# Autodesk Inventor assembly: Battery Rack Assembly
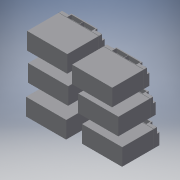
[picture p0: Inventor's stored thumbnail of the model, 180x180]
Saved by Autodesk Inventor 2019.4 (Build 234330000, 330)
## iProperties
Created: 2020-02-27
Part Number: Battery Rack Assembly
Document SubType Name: Assembly
Designer: admin
Author: admin
## Documents named in this file (2)
- C:\Users\admin\Desktop\FRC 2020 Engineering\GitHub\7738-2020\Pit Station Designs\battery rack\Battery Rack Assembly.iam
- C:\Users\admin\Desktop\FRC 2020 Engineering\GitHub\7738-2020\CAD\Battery.ipt
## Components (6 placed, 1 different names)
1. Battery:1 — Flush:1, Mate:1, Flush:5
2. Battery:2 — Flush:3, Mate:4, Flush:5
3. Battery:3 — Flush:3, Flush:4, Mate:3, Mate:4
4. Battery:4 — Flush:1, Flush:2, Mate:1, Mate:2
5. Battery:5 — Flush:4, Mate:3, Mate:5
6. Battery:6 — Flush:2, Mate:2, Mate:5
## Relationships (10: Flush 5, Mate 5)
- Flush:1: Battery:1 ↔ Battery:4
- Flush:2: Battery:4 ↔ Battery:6
- Flush:3: Battery:2 ↔ Battery:3
- Flush:4: Battery:3 ↔ Battery:5
- Mate:1 (50 mm): Battery:1 ↔ Battery:4
- Mate:2 (50 mm): Battery:4 ↔ Battery:6
- Mate:3 (50 mm): Battery:3 ↔ Battery:5
- Mate:4 (50 mm): Battery:2 ↔ Battery:3
- Mate:5 (50 mm): Battery:5 ↔ Battery:6
- Flush:5: Battery:1 ↔ Battery:2
